# Autodesk Inventor assembly: Assembly_Cube_empty_IM_v3
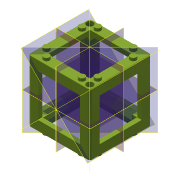
[picture p0: Inventor's stored thumbnail of the model, 180x180]
Saved by Autodesk Inventor 2022 (Build 260153000, 153)
## iProperties
Created: 2020-03-27
Part Number: Assembly_Cube_empty_IM_v3
Document SubType Name: Assembly
Designer: B
Mass: 22.3092 g
Surface Area: 188.369 cm^2
Volume: 22.3092 cm^3
Density: 1 g/cm^3
Author: B
## Documents named in this file (2)
- C:\Users\diederichbenedict\Dropbox\Dokumente\Promotion\PROJECTS\openUC2-CAD\INVENTOR\Assembly_Cube_empty_IM_v3.iam
- C:\Users\diederichbenedict\Dropbox\Dokumente\Promotion\PROJECTS\openUC2-CAD\INVENTOR\10_Cube_1x1_IM.ipt
## Components (2 placed, 1 different names)
1. 10_Cube_1x1_IM:1 — Angle:1, Mate:2, Symmetry:1, Symmetrie:2, Symmetrie:3, Symmetrie:4, Symmetrie:5, Symmetrie:6, Symmetrie:7, Symmetrie:8, Symmetrie:9
2. 10_Cube_1x1_IM:2 — Flush:1, Flush:2, Flush:3, Angle:1, Mate:2, Symmetry:1, Symmetrie:2, Symmetrie:3, Symmetrie:4, Symmetrie:5, Symmetrie:6, Symmetrie:7, Symmetrie:8, Symmetrie:9
## Relationships (18: Symmetry 9, Mate 5, Flush 3, Angle 1)
- Flush:1: 10_Cube_1x1_IM:2
- Flush:2: 10_Cube_1x1_IM:2
- Flush:3: 10_Cube_1x1_IM:2
- Angle:1 (0 deg): 10_Cube_1x1_IM:1 ↔ 10_Cube_1x1_IM:2
- Mate:2 (-50.1 mm): 10_Cube_1x1_IM:1 ↔ 10_Cube_1x1_IM:2
- Symmetry:1: 10_Cube_1x1_IM:1 ↔ 10_Cube_1x1_IM:2
- Symmetrie:2: 10_Cube_1x1_IM:1 ↔ 10_Cube_1x1_IM:2
- Symmetrie:3: 10_Cube_1x1_IM:1 ↔ 10_Cube_1x1_IM:2
- Symmetrie:4: 10_Cube_1x1_IM:1 ↔ 10_Cube_1x1_IM:2
- Symmetrie:5: 10_Cube_1x1_IM:1 ↔ 10_Cube_1x1_IM:2
- Symmetrie:6: 10_Cube_1x1_IM:1 ↔ 10_Cube_1x1_IM:2
- Symmetrie:7: 10_Cube_1x1_IM:1 ↔ 10_Cube_1x1_IM:2
- Passend:3 [Mate]
- Passend:4 [Mate]
- Symmetrie:8: 10_Cube_1x1_IM:1 ↔ 10_Cube_1x1_IM:2
- Symmetrie:9: 10_Cube_1x1_IM:1 ↔ 10_Cube_1x1_IM:2
- Passend:5 [Mate]
- Passend:6 [Mate]
